# Autodesk Inventor assembly: Head_neck_diagonal
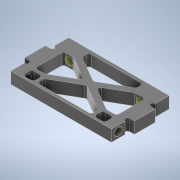
[picture p0: Inventor's stored thumbnail of the model, 180x180]
Saved by Autodesk Inventor 2022.3 (Build 263350000, 350)
## iProperties
Created: 2023-05-07
Part Number: Head_neck_diagonal
Document SubType Name: Assembly
Designer: Masato Kubotera
Author: Masato Kubotera
## Documents named in this file (3)
- C:\Users\Masato\Documents\Inventor\Inventor for CIT Brains\SUSTAINA-OP - mod\UpperBody\Head\Head_neck_diagonal.iam
- C:\Users\Masato\Documents\Inventor\Inventor for CIT Brains\SUSTAINA-OP - mod\UpperBody\Head\Head_neck_diagonal.ipt
- C:\Users\Masato\Documents\Inventor\Inventor for CIT Brains\SUSTAINA-OP - mod\ReadyMade\InsertNut\IRU-304S.ipt
## Components (5 placed, 2 different names)
1. Head_neck_diagonal:1 — フラッシュ:1, フラッシュ:2, フラッシュ:3, 挿入:1, 挿入:2, 挿入:3, 挿入:4
2. IRU-304S:1 — 挿入:1
3. IRU-304S:2 — 挿入:2
4. IRU-304S:3 — 挿入:3
5. IRU-304S:4 — 挿入:4
## Relationships (7: Insert 4, Flush 3)
- フラッシュ:1 [Flush]: Head_neck_diagonal:1
- フラッシュ:2 [Flush]: Head_neck_diagonal:1
- フラッシュ:3 [Flush]: Head_neck_diagonal:1
- 挿入:1 [Insert]: Head_neck_diagonal:1 ↔ IRU-304S:1
- 挿入:2 [Insert]: Head_neck_diagonal:1 ↔ IRU-304S:2
- 挿入:3 [Insert]: Head_neck_diagonal:1 ↔ IRU-304S:3
- 挿入:4 [Insert]: Head_neck_diagonal:1 ↔ IRU-304S:4
